# Autodesk Inventor assembly: Assembly1
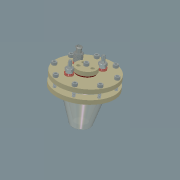
[picture p0: Inventor's stored thumbnail of the model, 180x180]
Saved by Autodesk Inventor 2016 (Build 200138000, 138)
## iProperties
Created: 2016-07-24
Part Number: Assembly1
Document SubType Name: Assembly
Designer: ashish
Author: ashish
## Documents named in this file (12)
- C:\BMBB 2015-2020\Bond lab\bioreactor design\Assembly1.iam
- C:\BMBB 2015-2020\Bond lab\bioreactor design\lid.ipt
- C:\BMBB 2015-2020\Bond lab\bioreactor design\gasket.ipt
- C:\BMBB 2015-2020\Bond lab\bioreactor design\washer.ipt
- C:\BMBB 2015-2020\Bond lab\bioreactor design\2844K130_NICKEL-PLTD BRASS BARBED VACUUM TUBE FITTING.ipt
- C:\BMBB 2015-2020\Bond lab\bioreactor design\51465K161_HIGH-STRENGTH QUICK-TURN TUBE COUPLING.ipt
- C:\BMBB 2015-2020\Bond lab\bioreactor design\15 ml cone.ipt
- C:\BMBB 2015-2020\Bond lab\bioreactor design\ring - Copy.ipt
- C:\BMBB 2015-2020\Bond lab\bioreactor design\100ml final\92196A150_18-8 STAINLESS STEEL SOCKET HEAD CAP SCREW.ipt
- C:\BMBB 2015-2020\Bond lab\bioreactor design\100ml final\92196A146_18-8 STAINLESS STEEL SOCKET HEAD CAP SCREW.ipt
- C:\BMBB 2015-2020\Bond lab\bioreactor design\Part5.ipt
- C:\BMBB 2015-2020\Bond lab\bioreactor design\ring.ipt
## Components (21 placed, 11 different names)
1. lid:1 — Rigid:1, Rotational:1, Rigid:2, Rigid:3, Insert:1, Insert:2, Insert:3, Rigid:5, Rotational:4, Rotational:5, Rotational:6, Rigid:6, Rotational:7, Rotational:8, Insert:4
2. gasket:1 — Rigid:1
3. washer:1 — Rotational:1, Rotational:3
4. washer:2 — Rigid:3, Rotational:2
5. washer:3 — Rigid:2, Rigid:4
6. 2844K130_NICKEL-PLTD BRASS BARBED VACUUM TUBE FITTING:1 — Rotational:3
7. 2844K130_NICKEL-PLTD BRASS BARBED VACUUM TUBE FITTING:2 — Rotational:2
8. 51465K161_HIGH-STRENGTH QUICK-TURN TUBE COUPLING:1 — Rigid:4
9. 15 ml cone:2 — Insert:1, Mate:1
10. ring - Copy:2 — Insert:2, Mate:1
11. 92196A150_18-8 STAINLESS STEEL SOCKET HEAD CAP SCREW:1 — Rotational:8
12. 92196A150_18-8 STAINLESS STEEL SOCKET HEAD CAP SCREW:2 — Rigid:6
13. 92196A150_18-8 STAINLESS STEEL SOCKET HEAD CAP SCREW:3 — Rotational:6
14. 92196A150_18-8 STAINLESS STEEL SOCKET HEAD CAP SCREW:4 — Rotational:5
15. 92196A150_18-8 STAINLESS STEEL SOCKET HEAD CAP SCREW:5 — Insert:3
16. 92196A150_18-8 STAINLESS STEEL SOCKET HEAD CAP SCREW:6 — Rotational:4
17. 92196A150_18-8 STAINLESS STEEL SOCKET HEAD CAP SCREW:7 — Rotational:7
18. 92196A150_18-8 STAINLESS STEEL SOCKET HEAD CAP SCREW:8 — Rigid:5
19. 92196A146_18-8 STAINLESS STEEL SOCKET HEAD CAP SCREW:1 — Insert:6
20. Part5:1 — Insert:4, Insert:5
21. ring:1 — Insert:5, Insert:6
## Relationships (21: RevoluteJoint 8, WeldJoint 6, Insert 6, Mate 1)
- Rigid:1 [WeldJoint]: lid:1 ↔ gasket:1
- Rotational:1 [RevoluteJoint]: lid:1 ↔ washer:1
- Rigid:2 [WeldJoint]: lid:1 ↔ washer:3
- Rigid:3 [WeldJoint]: lid:1 ↔ washer:2
- Rotational:2 [RevoluteJoint] (-12.7 mm): washer:2 ↔ 2844K130_NICKEL-PLTD BRASS BARBED VACUUM TUBE FITTING:2
- Rotational:3 [RevoluteJoint] (-12.7 mm): washer:1 ↔ 2844K130_NICKEL-PLTD BRASS BARBED VACUUM TUBE FITTING:1
- Rigid:4 [WeldJoint] (6.4262 mm): washer:3 ↔ 51465K161_HIGH-STRENGTH QUICK-TURN TUBE COUPLING:1
- Insert:1: lid:1 ↔ 15 ml cone:2
- Insert:2 (6.35 mm): lid:1 ↔ ring - Copy:2
- Insert:3: lid:1 ↔ 92196A150_18-8 STAINLESS STEEL SOCKET HEAD CAP SCREW:5
- Rigid:5 [WeldJoint]: lid:1 ↔ 92196A150_18-8 STAINLESS STEEL SOCKET HEAD CAP SCREW:8
- Rotational:4 [RevoluteJoint]: lid:1 ↔ 92196A150_18-8 STAINLESS STEEL SOCKET HEAD CAP SCREW:6
- Rotational:5 [RevoluteJoint]: lid:1 ↔ 92196A150_18-8 STAINLESS STEEL SOCKET HEAD CAP SCREW:4
- Rotational:6 [RevoluteJoint]: lid:1 ↔ 92196A150_18-8 STAINLESS STEEL SOCKET HEAD CAP SCREW:3
- Rigid:6 [WeldJoint]: lid:1 ↔ 92196A150_18-8 STAINLESS STEEL SOCKET HEAD CAP SCREW:2
- Rotational:7 [RevoluteJoint]: lid:1 ↔ 92196A150_18-8 STAINLESS STEEL SOCKET HEAD CAP SCREW:7
- Rotational:8 [RevoluteJoint]: lid:1 ↔ 92196A150_18-8 STAINLESS STEEL SOCKET HEAD CAP SCREW:1
- Mate:1: 15 ml cone:2 ↔ ring - Copy:2
- Insert:4: lid:1 ↔ Part5:1
- Insert:5: Part5:1 ↔ ring:1
- Insert:6 (-8.89 mm): 92196A146_18-8 STAINLESS STEEL SOCKET HEAD CAP SCREW:1 ↔ ring:1
